# Autodesk Inventor assembly: ASY MSC 201 BACK
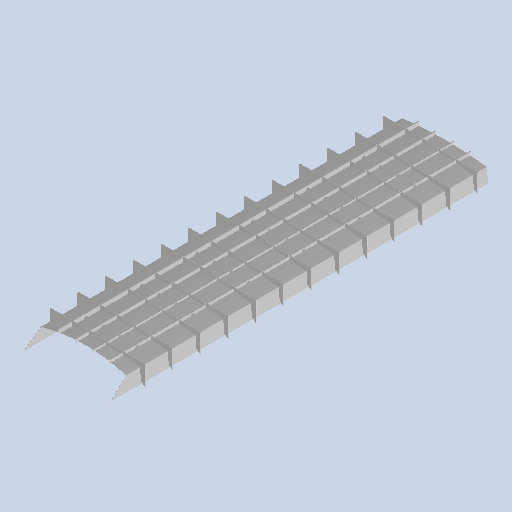
[picture p0: Inventor's stored thumbnail of the model, 512x512]
Saved by Autodesk Inventor 2025 (Build 290162010, 162A)
## iProperties
Created: 2024-07-19
Part Number: ASY MSC 201 BACK
Document SubType Name: Assembly
Designer: pokla
Author: pokla
## Documents named in this file (9)
- C:\Users\user\YandexDisk\домашниий пк\Inventor\Manturovo\Manturovo_Se-clar\ASY MSC 201 BACK.iam
- C:\Users\user\YandexDisk\домашниий пк\Inventor\Manturovo\Manturovo_Se-clar\MSC 033 sheet back basic.ipt
- C:\Users\user\YandexDisk\домашниий пк\Inventor\Manturovo\Manturovo_Se-clar\MSC 051 rib back.ipt
- C:\Users\user\YandexDisk\домашниий пк\Inventor\Manturovo\Manturovo_Se-clar\MSC 034 sheet back-neck.ipt
- C:\Users\user\YandexDisk\домашниий пк\Inventor\Manturovo\Manturovo_Se-clar\MSC 061 stringer back ^.ipt
- C:\Users\user\YandexDisk\домашниий пк\Inventor\Manturovo\Manturovo_Se-clar\MSC 062 stringer back ^^.ipt
- C:\Users\user\YandexDisk\домашниий пк\Inventor\Manturovo\Manturovo_Se-clar\MSC 0331 sheet back mould.ipt
- C:\Users\user\YandexDisk\домашниий пк\Inventor\Manturovo\Manturovo_Se-clar\MSC 061.1 stringer back ^.ipt
- C:\Users\user\YandexDisk\домашниий пк\Inventor\Manturovo\Manturovo_Se-clar\MSC 062.1 stringer back ^^.ipt
## Components (74 placed, 12 different names)
1. MSC 033 sheet back basic:6 — Flush:3, Flush:4, Mate:2, Rigid:64, Mate:3, Mate:4, Flush:5
2. MSC 033 sheet back basic.ipt:3 — Mate:1, Flush:2, Tangent:2, Rigid:64, Rigid:65
3. MSC 033 sheet back basic.ipt:1 — Rigid:65, Rigid:66
4. MSC 033 sheet back basic.ipt:2 — Rigid:66, Rigid:67
5. MSC 034 sheet back-neck.ipt:1 — Rigid:69
6. MSC 033 sheet back basic.ipt:5 — Rigid:68, Rigid:69
7. MSC 033 sheet back basic.ipt:4 — Rigid:67, Rigid:68
8. MSC 061 stringer back ^.ipt:1 — Rigid:75, Rigid:76, Rigid:80
9. MSC 061 stringer back ^.ipt:2 — Rigid:77, Rigid:81
10. MSC 062 stringer back ^^.ipt:2 — Rigid:78, Rigid:82
11. MSC 062 stringer back ^^.ipt:1 — Rigid:79, Rigid:83
12. MSC 051 rib back.ipt:4 — Rigid:70, Mate:3, Rigid:73, Flush:5
13. MSC 051 rib back.ipt:5 — Rigid:70, Mate:4
14. MSC 061.1 stringer back ^:1 — Rigid:80
15. MSC 061.1 stringer back ^:2 — Rigid:81
16. MSC 062.1 stringer back ^^:1 — Rigid:82
17. MSC 062.1 stringer back ^^:2 — Rigid:83
18. MSC 0331 sheet back mould:1 — Mate:1, Flush:2, Tangent:2, Rigid:22, Rigid:23
19. MSC 0331 sheet back mould:2 — Rigid:22, Rigid:25
20. MSC 0331 sheet back mould:3 — Rigid:23, Rigid:24
21. MSC 0331 sheet back mould:4 — Rigid:24
22. MSC 0331 sheet back mould:5 — Rigid:25, Rigid:27
23. MSC 0331 sheet back mould:6 — Rigid:27
24. MSC 0331 sheet back mould:7 — Rigid:31
25. MSC 0331 sheet back mould:8 — Rigid:31
26. MSC 0331 sheet back mould:9
27. MSC 0331 sheet back mould:10
28. MSC 0331 sheet back mould:11 — Rigid:33
29. MSC 0331 sheet back mould:12 — Rigid:33
30. MSC 0331 sheet back mould:13
31. MSC 051 rib back.ipt:2 — Rigid:73, Rigid:74, Rigid:78
32. MSC 051 rib back.ipt:3 — Rigid:74, Rigid:77, Rigid:79
33. MSC 051 rib back:8 — Rigid:75
34. MSC 051 rib back:9
35. MSC 051 rib back:10
36. MSC 051 rib back:11
37. MSC 051 rib back:12
38. MSC 051 rib back:13
39. MSC 051 rib back:14
40. MSC 051 rib back:15
41. MSC 051 rib back:16
42. MSC 051 rib back:17
43. MSC 051 rib back:18
44. MSC 051 rib back:19
45. MSC 051 rib back:20
46. MSC 051 rib back:21
47. MSC 051 rib back:22
48. MSC 051 rib back:23
49. MSC 051 rib back:24
50. MSC 051 rib back:25
51. MSC 051 rib back:26
52. MSC 051 rib back:27
53. MSC 051 rib back:28
54. MSC 051 rib back:29
55. MSC 062 stringer back ^^.ipt:3
56. МОО 051 стрингер спина 1:6 — Rigid:76
57. MSC 061 stringer back ^.ipt:4
58. MSC 062 stringer back ^^.ipt:4
59. МОО 052 стрингер спина 2:6
60. МОО 051 стрингер спина 1:7
61. МОО 051 стрингер спина 1:8
62. МОО 052 стрингер спина 2:7
63. МОО 052 стрингер спина 2:8
64. МОО 051 стрингер спина 1:9
65. МОО 051 стрингер спина 1:10
66. МОО 052 стрингер спина 2:9
67. МОО 052 стрингер спина 2:10
68. МОО 051 стрингер спина 1:11
69. МОО 051 стрингер спина 1:12
70. МОО 052 стрингер спина 2:11
71. МОО 052 стрингер спина 2:12
72. МОО 051 стрингер спина 1:13
73. МОО 051 стрингер спина 1:14
74. МОО 052 стрингер спина 2:13
## Component patterns: (12 elements, first: MSC 051 rib back.ipt:2 + MSC 051 rib back.ipt:3), (5 elements, first: MSC 062 stringer back ^^.ipt:3 + МОО 051 стрингер спина 1:6 + MSC 061 stringer back ^.ipt:4 + MSC 062 stringer back ^^.ipt:4)
## Relationships (42: WeldJoint 33, Mate 4, Flush 4, Tangent 1)
- [WeldJoint]: MSC 061 stringer back ^.ipt:2 ↔ MSC 061 stringer back ^.ipt:4
- [WeldJoint]: MSC 062 stringer back ^^.ipt:2 ↔ MSC 062 stringer back ^^.ipt:3
- [WeldJoint]: MSC 062 stringer back ^^.ipt:1 ↔ MSC 062 stringer back ^^.ipt:4
- Mate:1: MSC 033 sheet back basic.ipt:3 ↔ MSC 0331 sheet back mould:1
- Flush:2 (248.5 mm): MSC 033 sheet back basic.ipt:3 ↔ MSC 0331 sheet back mould:1
- Tangent:2: MSC 033 sheet back basic.ipt:3 ↔ MSC 0331 sheet back mould:1
- Rigid:22 [WeldJoint] (497 mm): MSC 0331 sheet back mould:1 ↔ MSC 0331 sheet back mould:2
- Rigid:23 [WeldJoint] (497 mm): MSC 0331 sheet back mould:1 ↔ MSC 0331 sheet back mould:3
- Rigid:24 [WeldJoint] (497 mm): MSC 0331 sheet back mould:3 ↔ MSC 0331 sheet back mould:4
- Rigid:25 [WeldJoint] (497 mm): MSC 0331 sheet back mould:2 ↔ MSC 0331 sheet back mould:5
- [WeldJoint] (497 mm): MSC 0331 sheet back mould:6 ↔ MSC 0331 sheet back mould:7
- Rigid:27 [WeldJoint] (497 mm): MSC 0331 sheet back mould:5 ↔ MSC 0331 sheet back mould:6
- [WeldJoint] (497 mm): MSC 0331 sheet back mould:8 ↔ MSC 0331 sheet back mould:9
- [WeldJoint] (497 mm): MSC 0331 sheet back mould:10 ↔ MSC 0331 sheet back mould:11
- [WeldJoint] (497 mm): MSC 0331 sheet back mould:9 ↔ MSC 0331 sheet back mould:10
- Rigid:31 [WeldJoint] (497 mm): MSC 0331 sheet back mould:7 ↔ MSC 0331 sheet back mould:8
- [WeldJoint] (497 mm): MSC 0331 sheet back mould:12 ↔ MSC 0331 sheet back mould:13
- Rigid:33 [WeldJoint] (497 mm): MSC 0331 sheet back mould:11 ↔ MSC 0331 sheet back mould:12
- Flush:3: MSC 033 sheet back basic:6
- Flush:4: MSC 033 sheet back basic:6
- Mate:2: MSC 033 sheet back basic:6
- Rigid:64 [WeldJoint]: MSC 033 sheet back basic:6 ↔ MSC 033 sheet back basic.ipt:3
- Rigid:65 [WeldJoint]: MSC 033 sheet back basic.ipt:3 ↔ MSC 033 sheet back basic.ipt:1
- Rigid:66 [WeldJoint]: MSC 033 sheet back basic.ipt:1 ↔ MSC 033 sheet back basic.ipt:2
- Rigid:67 [WeldJoint]: MSC 033 sheet back basic.ipt:2 ↔ MSC 033 sheet back basic.ipt:4
- Rigid:68 [WeldJoint]: MSC 033 sheet back basic.ipt:5 ↔ MSC 033 sheet back basic.ipt:4
- Rigid:69 [WeldJoint]: MSC 034 sheet back-neck.ipt:1 ↔ MSC 033 sheet back basic.ipt:5
- Rigid:70 [WeldJoint] (-100 mm): MSC 051 rib back.ipt:4 ↔ MSC 051 rib back.ipt:5
- Mate:3: MSC 033 sheet back basic:6 ↔ MSC 051 rib back.ipt:4
- Mate:4: MSC 033 sheet back basic:6 ↔ MSC 051 rib back.ipt:5
- Rigid:73 [WeldJoint] (-490 mm): MSC 051 rib back.ipt:4 ↔ MSC 051 rib back.ipt:2
- Rigid:74 [WeldJoint] (-100 mm): MSC 051 rib back.ipt:2 ↔ MSC 051 rib back.ipt:3
- Rigid:75 [WeldJoint] (2 mm): MSC 061 stringer back ^.ipt:1 ↔ MSC 051 rib back:8
- Flush:5 (245 mm): MSC 033 sheet back basic:6 ↔ MSC 051 rib back.ipt:4
- Rigid:76 [WeldJoint]: MSC 061 stringer back ^.ipt:1 ↔ МОО 051 стрингер спина 1:6
- Rigid:77 [WeldJoint]: MSC 061 stringer back ^.ipt:2 ↔ MSC 051 rib back.ipt:3
- Rigid:78 [WeldJoint] (2 mm): MSC 062 stringer back ^^.ipt:2 ↔ MSC 051 rib back.ipt:2
- Rigid:79 [WeldJoint]: MSC 062 stringer back ^^.ipt:1 ↔ MSC 051 rib back.ipt:3
- Rigid:80 [WeldJoint]: MSC 061 stringer back ^.ipt:1 ↔ MSC 061.1 stringer back ^:1
- Rigid:81 [WeldJoint]: MSC 061 stringer back ^.ipt:2 ↔ MSC 061.1 stringer back ^:2
- Rigid:82 [WeldJoint]: MSC 062 stringer back ^^.ipt:2 ↔ MSC 062.1 stringer back ^^:1
- Rigid:83 [WeldJoint]: MSC 062 stringer back ^^.ipt:1 ↔ MSC 062.1 stringer back ^^:2
## Named parameters: d42_d41 = 497 mm, d44_d41 = 497 mm, d45_d42_d41 = 497 mm, d46_d43 = 497 mm, d48_d45_d42_d41 = 497 mm
